# Autodesk Inventor assembly: am14u3LongWithLiftMechanism
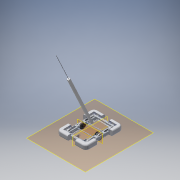
[picture p0: Inventor's stored thumbnail of the model, 180x180]
Saved by Autodesk Inventor 2018.2 (Build 222227000, 227)
## iProperties
Created: 2018-01-10
Part Number: am14u3LongWithLiftMechanism
Document SubType Name: Assembly
Designer: steele
Author: steele
## Documents named in this file (4)
- D:\snobotics\CAD-Development\robSteele\2018-FRC\am14u3LongWithLiftMechanism.iam
- D:\snobotics\CAD-Development\robSteele\2018-FRC\AM14U3 Long with Bumper\DB_DriveBaseLong_AM14U3_Bumpers and Battery Tray.iam
- D:\snobotics\CAD-Development\robSteele\2018-FRC\AluminumTubing\2x2x1_8_tubeForLift.ipt
- D:\snobotics\CAD-Development\robSteele\2018-FRC\RobotLiftMechanism\airCylinder30inStroke.ipt
## Components (3 placed, 3 different names)
1. DB_DriveBaseLong_AM14U3_Bumpers and Battery Tray:1 [sub-assembly] — Mate:1, Angle:1, Mate:2, Mate:3
2. 2x2x1_8_tubeForLift:1 — Mate:1, Angle:1, Mate:2, Mate:3, Insert:1
3. airCylinder30inStroke:1 — Insert:1
## Relationships (5: Mate 3, Angle 1, Insert 1)
- Mate:1: DB_DriveBaseLong_AM14U3_Bumpers and Battery Tray:1 ↔ 2x2x1_8_tubeForLift:1
- Angle:1 (25 deg): DB_DriveBaseLong_AM14U3_Bumpers and Battery Tray:1 ↔ 2x2x1_8_tubeForLift:1
- Mate:2: DB_DriveBaseLong_AM14U3_Bumpers and Battery Tray:1 ↔ 2x2x1_8_tubeForLift:1
- Mate:3 (-609.6 mm): DB_DriveBaseLong_AM14U3_Bumpers and Battery Tray:1 ↔ 2x2x1_8_tubeForLift:1
- Insert:1: 2x2x1_8_tubeForLift:1 ↔ airCylinder30inStroke:1
